# Autodesk Inventor assembly: Z-axis Assembly
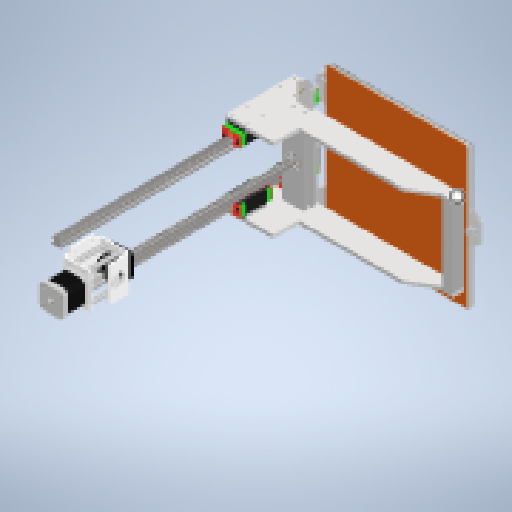
[picture p0: Inventor's stored thumbnail of the model, 512x512]
Saved by Autodesk Inventor 2024 (Build 280153000, 153)
## iProperties
Created: 2024-12-16
Part Number: Z-axis Assembly
Document SubType Name: Assembly
Designer: Ishaan
Author: Ishaan
## Documents named in this file (21)
- E:\Projects\Axiom--IDEX-3D-Printer\CAD\02 - Z-axis\Z-axis Assembly.iam
- E:\Projects\Axiom--IDEX-3D-Printer\CAD\01 - Frame\4080 Z-Rail.ipt
- E:\Projects\Axiom--IDEX-3D-Printer\CAD\02 - Z-axis\Z-Axis Drive Mount.ipt
- E:\Projects\Axiom--IDEX-3D-Printer\CAD\00 - COTS Components\FK10\FK10-C5\FK10-C5\FK10-C5.iam
- E:\Projects\Axiom--IDEX-3D-Printer\CAD\00 - COTS Components\SFU1204 Ballscrew\1204 Ballscrew.ipt
- E:\Projects\Axiom--IDEX-3D-Printer\CAD\00 - COTS Components\FK10\FK10-C5\Гайка М10х1\Гайка М10х1.iam
- E:\Projects\Axiom--IDEX-3D-Printer\CAD\00 - COTS Components\NEMA 17 - Z-Axis Long\NEMA 17 Z-axis Long.ipt
- E:\Projects\Axiom--IDEX-3D-Printer\CAD\00 - COTS Components\5x8 Shaft Coupler\Flexible Coupling 5mm x 8mm.ipt
- E:\Projects\Axiom--IDEX-3D-Printer\CAD\00 - COTS Components\60mm M5 Standoff\60mm M5 Standoff.ipt
- E:\Projects\Axiom--IDEX-3D-Printer\CAD\00 - COTS Components\HGR15 Z-Axis Rail\HGR15-R-700mm\HGR15-R-700mm.iam
- E:\Projects\Axiom--IDEX-3D-Printer\CAD\00 - COTS Components\HGH15CA Carriage Block\HGH15CA Hiwin Linear block by proma\HGH15CA Hiwin Linear block by proma.ipt
- E:\Projects\Axiom--IDEX-3D-Printer\CAD\02 - Z-axis\Z-Axis Bed Plates.ipt
- E:\Projects\Axiom--IDEX-3D-Printer\CAD\02 - Z-axis\2020 Bed Front Extrusion.ipt
- E:\Projects\Axiom--IDEX-3D-Printer\CAD\02 - Z-axis\2040 Bed Rear Extrusion.ipt
- E:\Projects\Axiom--IDEX-3D-Printer\CAD\02 - Z-axis\Z-Axis Nut and Bed Plate RevII.ipt
- E:\Projects\Axiom--IDEX-3D-Printer\CAD\00 - COTS Components\1204 Ballscrew Nut\Ballscrew nut 1204 by proma\Ballscrew nut 1204 by proma.ipt
- E:\Projects\Axiom--IDEX-3D-Printer\CAD\02 - Z-axis\Bed Heater.ipt
- E:\Projects\Axiom--IDEX-3D-Printer\CAD\02 - Z-axis\Bed Magnet.ipt
- E:\Projects\Axiom--IDEX-3D-Printer\CAD\02 - Z-axis\PEI Bed Surface.ipt
- E:\Projects\Axiom--IDEX-3D-Printer\CAD\02 - Z-axis\Print Bed Washers.ipt
- E:\Projects\Axiom--IDEX-3D-Printer\CAD\02 - Z-axis\Print Bed.ipt
## Components (30 placed, 20 different names)
1. Z-Axis Drive Mount:1 — Mate:1, Flush:1, Flush:2, Insert:1, Insert:2, Insert:5, Insert:6, Insert:8, Insert:9, Insert:10, Insert:11
2. 4080 Z-rail:1 — Mate:1, Flush:1, Flush:2, Mate:2, Mate:3, Flush:3, Mate:4, Mate:5, Flush:5, Flush:7, Flush:8
3. FK10-C5:1 [sub-assembly] — Insert:1, Insert:2, Insert:3, Insert:4, Mate:18
4. 1204 Ballscrew:1 — Insert:3, Mate:11, Flush:15
5. Гайка М10х1:1 [sub-assembly] — Insert:4
6. NEMA 17 Z-axis Long:1 — Insert:5, Insert:6, Insert:7
7. Flexible Coupling 5mm x 8mm:1 — Insert:7
8. 60mm M5 Standoff:1 — Insert:8
9. 60mm M5 Standoff:2 — Insert:9
10. 60mm M5 Standoff:3 — Insert:10
11. 60mm M5 Standoff:4 — Insert:11
12. HGR15-R-700mm:1 [sub-assembly] — Mate:2, Mate:3, Flush:3, Flush:4, Mate:6, Mate:7
13. HGR15-R-700mm:2 [sub-assembly] — Mate:4, Mate:5, Flush:4, Mate:8, Mate:9
14. HGH15CA Hiwin Linear block by proma:1 — Mate:6, Flush:5, Flush:6, Insert:14, Insert:15
15. HGH15CA Hiwin Linear block by proma:2 — Mate:7, Flush:6, Insert:12, Insert:13
16. HGH15CA Hiwin Linear block by proma:3 — Mate:8, Flush:7, Insert:18, Insert:19
17. HGH15CA Hiwin Linear block by proma:4 — Mate:9, Flush:8, Insert:16, Insert:17
18. Z-Axis Bed Plates:1 — Insert:12, Insert:13, Insert:14, Insert:15, Insert:20, Angle:1, Insert:24, Insert:25
19. Z-Axis Bed Plates:2 — Insert:16, Insert:17, Insert:18, Insert:19, Insert:21, Insert:22, Insert:23
20. 2020 Bed Front Extrusion:1 — Insert:20, Insert:21, Angle:1, Angle:2, Mate:12, Mate:16
21. 2040 Bed Rear Extrusion:1 — Insert:22, Insert:23, Insert:24, Insert:25, Mate:10
22. Z-Axis Nut and Bed Plate RevII:1 — Mate:10, Mate:11, Angle:2, Insert:26, Insert:27, Mate:17
23. Ballscrew nut 1204 by proma:1 — Insert:26, Insert:27, Flush:15, Mate:18
24. Bed Heater:1 — Mate:15, Flush:13, Flush:14
25. Bed Magnet:1 — Mate:13, Flush:9, Flush:10, Mate:14, Flush:11, Flush:12
26. PEI Bed Surface:1 — Mate:14, Flush:11, Flush:12
27. Print Bed Washers:1 — Insert:28, Mate:16
28. Print Bed:1 — Mate:12, Mate:13, Flush:9, Flush:10, Mate:15, Flush:13, Flush:14, Insert:28, Insert:29, Insert:30, Mate:17
29. Print Bed Washers:2 — Insert:29
30. Print Bed Washers:3 — Insert:30
## Relationships (65: Insert 30, Mate 18, Flush 15, Angle 2)
- Mate:1: Z-Axis Drive Mount:1 ↔ 4080 Z-rail:1
- Flush:1 (10 mm): Z-Axis Drive Mount:1 ↔ 4080 Z-rail:1
- Flush:2 (2 mm): Z-Axis Drive Mount:1 ↔ 4080 Z-rail:1
- Insert:1: Z-Axis Drive Mount:1 ↔ FK10-C5:1
- Insert:2: Z-Axis Drive Mount:1 ↔ FK10-C5:1
- Insert:3: FK10-C5:1 ↔ 1204 Ballscrew:1
- Insert:4: FK10-C5:1 ↔ Гайка М10х1:1
- Insert:5: Z-Axis Drive Mount:1 ↔ NEMA 17 Z-axis Long:1
- Insert:6: Z-Axis Drive Mount:1 ↔ NEMA 17 Z-axis Long:1
- Insert:7: NEMA 17 Z-axis Long:1 ↔ Flexible Coupling 5mm x 8mm:1
- Insert:8: Z-Axis Drive Mount:1 ↔ 60mm M5 Standoff:1
- Insert:9: Z-Axis Drive Mount:1 ↔ 60mm M5 Standoff:2
- Insert:10: Z-Axis Drive Mount:1 ↔ 60mm M5 Standoff:3
- Insert:11: Z-Axis Drive Mount:1 ↔ 60mm M5 Standoff:4
- Mate:2 (-10 mm): 4080 Z-rail:1 ↔ HGR15-R-700mm:1
- Mate:3: 4080 Z-rail:1 ↔ HGR15-R-700mm:1
- Flush:3 (-10 mm): 4080 Z-rail:1 ↔ HGR15-R-700mm:1
- Mate:4 (-10 mm): 4080 Z-rail:1 ↔ HGR15-R-700mm:2
- Mate:5: 4080 Z-rail:1 ↔ HGR15-R-700mm:2
- Flush:4: HGR15-R-700mm:1 ↔ HGR15-R-700mm:2
- Mate:6: HGR15-R-700mm:1 ↔ HGH15CA Hiwin Linear block by proma:1
- Flush:5 (28 mm): 4080 Z-rail:1 ↔ HGH15CA Hiwin Linear block by proma:1
- Mate:7: HGR15-R-700mm:1 ↔ HGH15CA Hiwin Linear block by proma:2
- Flush:6: HGH15CA Hiwin Linear block by proma:1 ↔ HGH15CA Hiwin Linear block by proma:2
- Mate:8: HGR15-R-700mm:2 ↔ HGH15CA Hiwin Linear block by proma:3
- Flush:7 (28 mm): 4080 Z-rail:1 ↔ HGH15CA Hiwin Linear block by proma:3
- Mate:9: HGR15-R-700mm:2 ↔ HGH15CA Hiwin Linear block by proma:4
- Flush:8 (28 mm): 4080 Z-rail:1 ↔ HGH15CA Hiwin Linear block by proma:4
- Insert:12: HGH15CA Hiwin Linear block by proma:2 ↔ Z-Axis Bed Plates:1
- Insert:13: HGH15CA Hiwin Linear block by proma:2 ↔ Z-Axis Bed Plates:1
- Insert:14: HGH15CA Hiwin Linear block by proma:1 ↔ Z-Axis Bed Plates:1
- Insert:15: HGH15CA Hiwin Linear block by proma:1 ↔ Z-Axis Bed Plates:1
- Insert:16: HGH15CA Hiwin Linear block by proma:4 ↔ Z-Axis Bed Plates:2
- Insert:17: HGH15CA Hiwin Linear block by proma:4 ↔ Z-Axis Bed Plates:2
- Insert:18: HGH15CA Hiwin Linear block by proma:3 ↔ Z-Axis Bed Plates:2
- Insert:19: HGH15CA Hiwin Linear block by proma:3 ↔ Z-Axis Bed Plates:2
- Insert:20: Z-Axis Bed Plates:1 ↔ 2020 Bed Front Extrusion:1
- Insert:21: Z-Axis Bed Plates:2 ↔ 2020 Bed Front Extrusion:1
- Angle:1 (0 deg): Z-Axis Bed Plates:1 ↔ 2020 Bed Front Extrusion:1
- Insert:22: Z-Axis Bed Plates:2 ↔ 2040 Bed Rear Extrusion:1
- Insert:23: Z-Axis Bed Plates:2 ↔ 2040 Bed Rear Extrusion:1
- Insert:24: Z-Axis Bed Plates:1 ↔ 2040 Bed Rear Extrusion:1
- Insert:25: Z-Axis Bed Plates:1 ↔ 2040 Bed Rear Extrusion:1
- Mate:10: 2040 Bed Rear Extrusion:1 ↔ Z-Axis Nut and Bed Plate RevII:1
- Mate:11: 1204 Ballscrew:1 ↔ Z-Axis Nut and Bed Plate RevII:1
- Angle:2 (0 deg): 2020 Bed Front Extrusion:1 ↔ Z-Axis Nut and Bed Plate RevII:1
- Insert:26: Z-Axis Nut and Bed Plate RevII:1 ↔ Ballscrew nut 1204 by proma:1
- Insert:27: Z-Axis Nut and Bed Plate RevII:1 ↔ Ballscrew nut 1204 by proma:1
- Mate:12: 2020 Bed Front Extrusion:1 ↔ Print Bed:1
- Mate:13: Bed Magnet:1 ↔ Print Bed:1
- Flush:9 (1 mm): Bed Magnet:1 ↔ Print Bed:1
- Flush:10 (-1 mm): Bed Magnet:1 ↔ Print Bed:1
- Mate:14: Bed Magnet:1 ↔ PEI Bed Surface:1
- Flush:11: Bed Magnet:1 ↔ PEI Bed Surface:1
- Flush:12: Bed Magnet:1 ↔ PEI Bed Surface:1
- Mate:15: Bed Heater:1 ↔ Print Bed:1
- Flush:13 (2 mm): Bed Heater:1 ↔ Print Bed:1
- Flush:14 (-2 mm): Bed Heater:1 ↔ Print Bed:1
- Insert:28: Print Bed Washers:1 ↔ Print Bed:1
- Mate:16 (20 mm): 2020 Bed Front Extrusion:1 ↔ Print Bed Washers:1
- Insert:29: Print Bed:1 ↔ Print Bed Washers:2
- Insert:30: Print Bed:1 ↔ Print Bed Washers:3
- Mate:17: Z-Axis Nut and Bed Plate RevII:1 ↔ Print Bed:1
- Flush:15: 1204 Ballscrew:1 ↔ Ballscrew nut 1204 by proma:1
- Mate:18: FK10-C5:1 ↔ Ballscrew nut 1204 by proma:1
